# Autodesk Inventor assembly: Assembly2
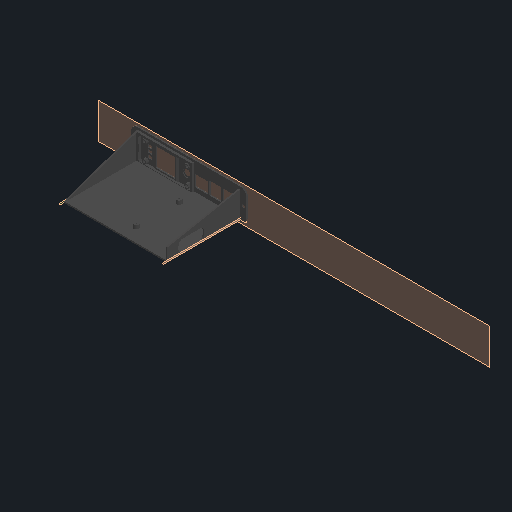
[picture p0: Inventor's stored thumbnail of the model, 512x512]
Saved by Autodesk Inventor 2026.2 (Build 302298010, 298A)
## iProperties
Created: 2026-03-25
Part Number: Assembly2
Document SubType Name: Assembly
Designer: usr
Author: usr
## Documents named in this file (3)
- C:\Users\usr\Documents\IP-TERMINAL\Assembly2.iam
- C:\Users\usr\Documents\IP-TERMINAL\RPI_HOUSING2.ipt
- C:\Users\usr\Documents\IP-TERMINAL\1.44lcd_cap_2.ipt
## Components (2 placed, 2 different names)
1. RPI_HOUSING2:1 — Mate:1, Flush:1, Flush:2
2. 1.44lcd_cap_2:1 — Mate:1, Flush:1, Flush:2
## Relationships (3: Flush 2, Mate 1)
- Mate:1: RPI_HOUSING2:1 ↔ 1.44lcd_cap_2:1
- Flush:1: RPI_HOUSING2:1 ↔ 1.44lcd_cap_2:1
- Flush:2: RPI_HOUSING2:1 ↔ 1.44lcd_cap_2:1
